# Autodesk Inventor assembly: SumirikiIsuka
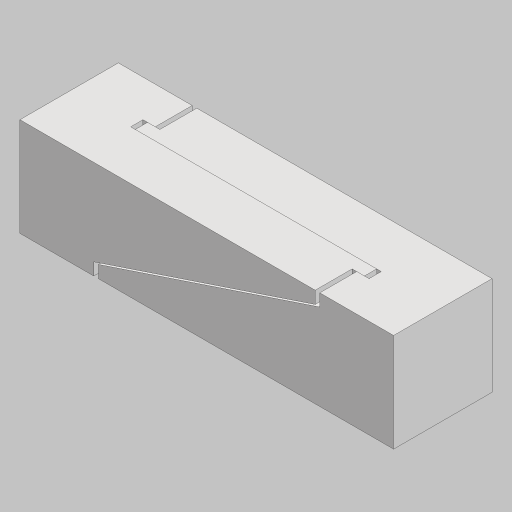
[picture p0: Inventor's stored thumbnail of the model, 512x512]
Saved by Autodesk Inventor 2023 (Build 270158000, 158)
## iProperties
Created: 2026-02-22
Part Number: SumirikiIsuka
Document SubType Name: Assembly
Designer: MARTIN MAESTRE
Author: MARTIN MAESTRE
## Documents named in this file (2)
- C:\Users\MARTIN MAESTRE\OneDrive - Universidad de los Andes\POSTGRADO\202610\MAESTRIA\PROBLEMA ESPECIAL\CADS\Fig5\SumirikiIsuka.iam
- C:\Users\MARTIN MAESTRE\OneDrive - Universidad de los Andes\POSTGRADO\202610\MAESTRIA\PROBLEMA ESPECIAL\CADS\Fig5\Hembra.ipt
## Components (2 placed, 1 different names)
1. Hembra:1 — Coincidencia:1, Nivelación:1, Coincidencia:2, Nivelación:2, Nivelación:3
2. Hembra:2 — Nivelación:2, Nivelación:3
## Relationships (5: Flush 3, Mate 2)
- Coincidencia:1 [Mate]: Hembra:1
- Nivelación:1 [Flush]: Hembra:1
- Coincidencia:2 [Mate]: Hembra:1
- Nivelación:2 [Flush]: Hembra:1 ↔ Hembra:2
- Nivelación:3 [Flush]: Hembra:1 ↔ Hembra:2
